# Autodesk Inventor assembly: 000ASS_Bo_banh_xe_02
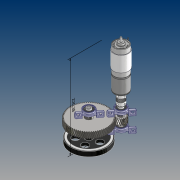
[picture p0: Inventor's stored thumbnail of the model, 180x180]
Saved by Autodesk Inventor 2021 (Build 250183000, 183)
## iProperties
Created: 2024-03-11
Part Number: 000ASS_Bo_banh_xe_02
Document SubType Name: Assembly
Designer: Admin
Author: Admin
## Documents named in this file (9)
- C:\Users\Admin\Desktop\DO_AN_TOT_NGHIEP_2024\Mechanical\Design_in_3D\Version_1\000ASS_Bo_banh_xe_02.iam
- C:\Users\Admin\Desktop\DO_AN_TOT_NGHIEP_2024\Mechanical\Design_in_3D\Version_1\01_Truc_01.ipt
- C:\Users\Admin\Desktop\DO_AN_TOT_NGHIEP_2024\Mechanical\Design_in_3D\Library\kp08-baering-with-housing-1.snapshot.4\KP08.iam
- C:\Users\Admin\Desktop\DO_AN_TOT_NGHIEP_2024\Mechanical\Design_in_3D\Library\planetary-gear-dc-motor-2.snapshot.1\Planetary Gear DC Motor\Planatary motor v1.ipt
- C:\Users\Admin\Desktop\DO_AN_TOT_NGHIEP_2024\Mechanical\Design_in_3D\Library\Banh_rang\Banh_rang_dan_01.ipt
- C:\Users\Admin\Desktop\DO_AN_TOT_NGHIEP_2024\Mechanical\Design_in_3D\Library\kh-p-n-i-m-m-2.snapshot.1\khop-noi-mem.ipt
- C:\Users\Admin\Desktop\DO_AN_TOT_NGHIEP_2024\Mechanical\Design_in_3D\Library\Banh_rang\Banh_rang_bi_dan_01.ipt
- C:\Users\Admin\Desktop\DO_AN_TOT_NGHIEP_2024\Mechanical\Design_in_3D\Library\banh-xe-robot-nhom-v5_2-1.snapshot.1\95mm phi 8 99g.ipt
- C:\Users\Admin\Desktop\DO_AN_TOT_NGHIEP_2024\Mechanical\Design_in_3D\Version_1\02_Truc_01.ipt
## Components (11 placed, 8 different names)
1. 01_Truc_01:1 — Mate:1, Mate:2, Mate:3, Mate:4, Flush:2, Mate:6
2. KP08:1 [sub-assembly] — Mate:2, Flush:1, Flush:6
3. KP08:2 [sub-assembly] — Mate:3, Flush:1, Flush:2, Flush:4, Flush:5, Mate:9
4. Planatary motor v1:1 — Mate:1, Mate:5
5. Spur Gear1:1 — Mate:4, Flush:3, Mate:9
6. khop-noi-mem:1 — Mate:5
7. Spur Gear2:1 — Mate:6, Flush:3, Mate:7, Mate:8, Mate:11
8. KP08:3 [sub-assembly] — Mate:7, Flush:4, Flush:5, Mate:10
9. KP08:4 [sub-assembly] — Mate:8, Flush:6, Flush:7
10. 95mm phi 8 99g:1 — Mate:10, Flush:8
11. 02_Truc_01:1 — Mate:11, Flush:7, Flush:8
## Relationships (19: Mate 11, Flush 8)
- Mate:1: 01_Truc_01:1 ↔ Planatary motor v1:1
- Mate:2: 01_Truc_01:1 ↔ KP08:1
- Mate:3: 01_Truc_01:1 ↔ KP08:2
- Flush:1: KP08:1 ↔ KP08:2
- Mate:4: 01_Truc_01:1 ↔ Spur Gear1:1
- Flush:2: 01_Truc_01:1 ↔ KP08:2
- Mate:5: Planatary motor v1:1 ↔ khop-noi-mem:1
- Mate:6 (59.88 mm): 01_Truc_01:1 ↔ Spur Gear2:1
- Flush:3: Spur Gear1:1 ↔ Spur Gear2:1
- Mate:7: Spur Gear2:1 ↔ KP08:3
- Flush:4: KP08:2 ↔ KP08:3
- Flush:5: KP08:2 ↔ KP08:3
- Mate:8: Spur Gear2:1 ↔ KP08:4
- Flush:6: KP08:1 ↔ KP08:4
- Mate:9 (3 mm): KP08:2 ↔ Spur Gear1:1
- Mate:10: KP08:3 ↔ 95mm phi 8 99g:1
- Mate:11: Spur Gear2:1 ↔ 02_Truc_01:1
- Flush:7: KP08:4 ↔ 02_Truc_01:1
- Flush:8: 95mm phi 8 99g:1 ↔ 02_Truc_01:1
